# Autodesk Inventor assembly: skatebaselat
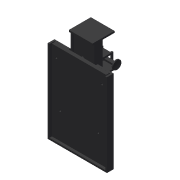
[picture p0: Inventor's stored thumbnail of the model, 180x180]
Saved by Autodesk Inventor 2021 Beta2 (Build 250156000, 156) ContinuousBuild 0
## iProperties
Created: 2002-04-25
Part Number: skatebaselat
Document SubType Name: Assembly
Designer: Administrator
Control State: 0
Master: False
Checked Out: False
Shininess: 64.0
Length Units: 11272
Angle Units: 11279
Time Units: 11290
Mass Units: 11286
Length Display Precision: 3
Angle Display Precision: 2
Density: 0.0
Volumn: 0.0
Area: 0.0
PropertySet Name: Model Information
Author: Administrator
## Documents named in this file (6)
- C:\Autodesk Inventor 2021 Intro Practice Files\skatebaselat.iam
- C:\Autodesk Inventor 2021 Intro Practice Files\staticplate.ipt
- C:\Autodesk Inventor 2021 Intro Practice Files\baseplate.ipt
- C:\Autodesk Inventor 2021 Intro Practice Files\lock.ipt
- C:\Autodesk Inventor 2021 Intro Practice Files\lock_MIR.ipt
- C:\Autodesk Inventor 2021 Intro Practice Files\slidelat.ipt
## Components (5 placed, 5 different names)
1. baseplate:1 — Insert:1, Mate:1
2. staticplate:1 — Insert:1, Mate:1, Mate:2, Insert:2, Flush:1, Mate:3, Mate:4
3. slidelat:1 — Flush:1, Mate:3, Mate:4
4. lock:1 — Mate:2, Insert:2
5. lock_MIR:1
## Relationships (7: Mate 4, Insert 2, Flush 1)
- Insert:1: baseplate:1 ↔ staticplate:1
- Mate:1: baseplate:1 ↔ staticplate:1
- Mate:2: staticplate:1 ↔ lock:1
- Insert:2: staticplate:1 ↔ lock:1
- Flush:1: staticplate:1 ↔ slidelat:1
- Mate:3 (25.4 mm): staticplate:1 ↔ slidelat:1
- Mate:4 (2.54 mm): staticplate:1 ↔ slidelat:1
